# Autodesk Inventor assembly: ENSAMBLADO DEL CUERPO
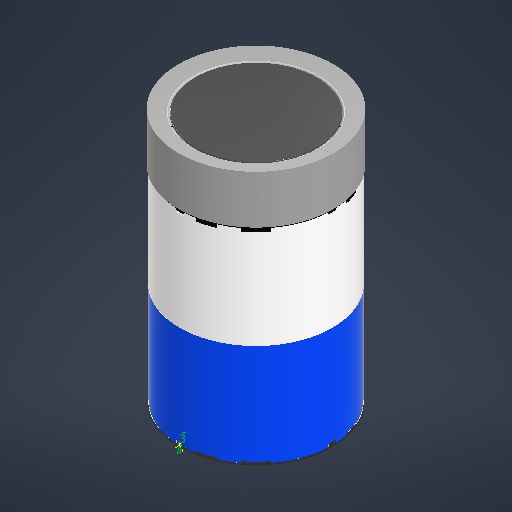
[picture p0: Inventor's stored thumbnail of the model, 512x512]
Saved by Autodesk Inventor 2026.1 (Build 301233020, 233B)
## iProperties
Created: 2026-05-13
Part Number: ENSAMBLADO DEL CUERPO
Document SubType Name: Assembly
Designer: USUARIO
Author: USUARIO
## Documents named in this file (8)
- C:\Users\USUARIO\Pictures\PROYECT INOVATION\ENSAMBLADO DEL CUERPO.iam
- C:\Users\USUARIO\Pictures\PROYECT INOVATION\P.BASE_4.ipt
- C:\Users\USUARIO\Pictures\PROYECT INOVATION\Cuerpo 1.ipt
- C:\Users\USUARIO\Pictures\PROYECT INOVATION\CUERPO 2.ipt
- C:\Users\USUARIO\Pictures\PROYECT INOVATION\TAPA DEL CUERPO.ipt
- C:\Users\USUARIO\Pictures\PROYECT INOVATION\bASE DEL PRIEMR SERVO.ipt
- C:\Users\USUARIO\Pictures\PROYECT INOVATION\pieza del platillo complemento.ipt
- C:\Users\USUARIO\Pictures\PROYECT INOVATION\Platillo.ipt
## Components (22 placed, 7 different names)
1. P.BASE_4:1 — Rígido:1, Rígido:7
2. P.BASE_4:2 — Rígido:1, Rígido:2
3. P.BASE_4:3 — Rígido:2, Rígido:3
4. P.BASE_4:4 — Rígido:3
5. Cuerpo 1:1 — Rígido:4
6. Cuerpo 1:2 — Rígido:5, Rígido:6, Rígido:7
7. Cuerpo 1:3 — Rígido:4, Rígido:5, Rígido:11
8. Cuerpo 1:4 — Rígido:6
9. CUERPO 2:1 — Rígido:8, Rígido:9, Rígido:11
10. CUERPO 2:2 — Rígido:8, Rígido:10
11. CUERPO 2:3 — Rígido:9, Rígido:15
12. CUERPO 2:4 — Rígido:10
13. TAPA DEL CUERPO:1 — Rígido:13
14. TAPA DEL CUERPO:2 — Rígido:12, Rígido:13, Rígido:16
15. TAPA DEL CUERPO:3 — Rígido:14, Rígido:15, De rotación:1
16. TAPA DEL CUERPO:4 — Rígido:12, Rígido:14
17. bASE DEL PRIEMR SERVO:1 — Rígido:16
18. pieza del platillo complemento:1 — Rígido:17, Rígido:18, Rígido:20
19. pieza del platillo complemento:2 — Rígido:18
20. pieza del platillo complemento:3 — Rígido:19
21. pieza del platillo complemento:4 — Rígido:17, Rígido:19, De rotación:1
22. Platillo:1 — Rígido:20
## Relationships (21: WeldJoint 20, RevoluteJoint 1)
- Rígido:1 [WeldJoint]: P.BASE_4:1 ↔ P.BASE_4:2
- Rígido:2 [WeldJoint]: P.BASE_4:2 ↔ P.BASE_4:3
- Rígido:3 [WeldJoint]: P.BASE_4:3 ↔ P.BASE_4:4
- Rígido:4 [WeldJoint]: Cuerpo 1:1 ↔ Cuerpo 1:3
- Rígido:5 [WeldJoint]: Cuerpo 1:2 ↔ Cuerpo 1:3
- Rígido:6 [WeldJoint]: Cuerpo 1:2 ↔ Cuerpo 1:4
- Rígido:7 [WeldJoint]: P.BASE_4:1 ↔ Cuerpo 1:2
- Rígido:8 [WeldJoint]: CUERPO 2:1 ↔ CUERPO 2:2
- Rígido:9 [WeldJoint]: CUERPO 2:1 ↔ CUERPO 2:3
- Rígido:10 [WeldJoint]: CUERPO 2:2 ↔ CUERPO 2:4
- Rígido:11 [WeldJoint]: Cuerpo 1:3 ↔ CUERPO 2:1
- Rígido:12 [WeldJoint]: TAPA DEL CUERPO:2 ↔ TAPA DEL CUERPO:4
- Rígido:13 [WeldJoint]: TAPA DEL CUERPO:1 ↔ TAPA DEL CUERPO:2
- Rígido:14 [WeldJoint]: TAPA DEL CUERPO:3 ↔ TAPA DEL CUERPO:4
- Rígido:15 [WeldJoint]: CUERPO 2:3 ↔ TAPA DEL CUERPO:3
- Rígido:16 [WeldJoint]: TAPA DEL CUERPO:2 ↔ bASE DEL PRIEMR SERVO:1
- Rígido:17 [WeldJoint]: pieza del platillo complemento:1 ↔ pieza del platillo complemento:4
- Rígido:18 [WeldJoint]: pieza del platillo complemento:1 ↔ pieza del platillo complemento:2
- Rígido:19 [WeldJoint]: pieza del platillo complemento:3 ↔ pieza del platillo complemento:4
- De rotación:1 [RevoluteJoint]: TAPA DEL CUERPO:3 ↔ pieza del platillo complemento:4
- Rígido:20 [WeldJoint]: pieza del platillo complemento:1 ↔ Platillo:1
